# Autodesk Inventor assembly: Z18936-A FULL ASSEMBLY
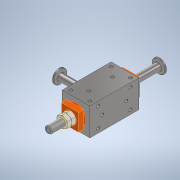
[picture p0: Inventor's stored thumbnail of the model, 180x180]
Saved by Autodesk Inventor 2021 (Build 250183000, 183)
## iProperties
Company: BROOKHAVEN NATIONAL LABORATORY
Created: 2019-11-05
Part Number: Z18936-A FULL ASSEMBLY
Description: ROTATING WATER JOINT SHAFT ASSEMBLY
Document SubType Name: Assembly
Designer: Work
Title: C:\Users\zconway\Documents\Inventor\HPR\Rotating Water Joint\Z18936-A FULL ASSEMBLY.stp
Author: zconway
Revision Number: 00
Sending System: Autodesk Inventor 2018
Preprocessor: ST-DEVELOPER v16.13
## Documents named in this file (9)
- C:\Users\Work\OneDrive - Brookhaven National Laboratory\Daniels, William intern HPR station\Arm\Z18936-A FULL ASSEMBLY.iam
- C:\Users\Work\OneDrive - Brookhaven National Laboratory\Daniels, William intern HPR station\Arm\Z18936-H HOUSING WELDMENT.iam
- C:\Users\Work\OneDrive - Brookhaven National Laboratory\Daniels, William intern HPR station\Arm\Z18936-S SHAFT ASSEMBLY.iam
- C:\Users\Work\OneDrive - Brookhaven National Laboratory\Daniels, William intern HPR station\Arm\Z18936-N1 COMPRESSION NUT.ipt
- C:\Users\Work\OneDrive - Brookhaven National Laboratory\Daniels, William intern HPR station\Arm\91907A140_TITANIUM THIN HEX NUT.ipt
- C:\Users\Work\OneDrive - Brookhaven National Laboratory\Daniels, William intern HPR station\Arm\8504A164_CORROSION-RESISTANT PRESS-FIT DRILL BUSHING.ipt
- C:\Users\Work\OneDrive - Brookhaven National Laboratory\Daniels, William intern HPR station\Arm\Z18936-B2 Shaft Gasket.ipt
- C:\Users\Work\OneDrive - Brookhaven National Laboratory\Daniels, William intern HPR station\Arm\Z18936-B1 THRUST PLATE.ipt
- C:\Users\Work\OneDrive - Brookhaven National Laboratory\Daniels, William intern HPR station\Arm\5908K150_ULTRA-CORROSION-RESISTANT SS BALL BEARING.ipt
## Components (13 placed, 8 different names)
1. Z18936-H HOUSING WELDMENT:1 [sub-assembly] — Rigid:5, Rigid:8, Rigid:12
2. Z18936-S SHAFT ASSEMBLY:1 [sub-assembly] — Rigid:7
3. Z18936-N1 COMPRESSION NUT:1 — Rigid:8
4. Z18936-N1 COMPRESSION NUT:2 — Rigid:5
5. 91907A140_TITANIUM THIN HEX NUT:1 — Rigid:3, Rigid:4
6. 91907A140_TITANIUM THIN HEX NUT:2 — Rigid:4
7. 8504A164_CORROSION-RESISTANT PRESS-FIT DRILL BUSHING:1 — Rigid:2, Rigid:3
8. Z18936-B2 Shaft Gasket:1 — Rigid:10, Rigid:11, Rigid:12
9. Z18936-B2 Shaft Gasket:2 — Rigid:9, Rigid:11
10. Z18936-B1 THRUST PLATE:1 — Rigid:6, Rigid:10
11. Z18936-B1 THRUST PLATE:2 — Rigid:1, Rigid:9
12. 5908K150_ULTRA-CORROSION-RESISTANT SS BALL BEARING:1 — Rigid:6, Rigid:7
13. 5908K150_ULTRA-CORROSION-RESISTANT SS BALL BEARING:2 — Rigid:1, Rigid:2
## Relationships (12: WeldJoint 12)
- Rigid:1 [WeldJoint]: Z18936-B1 THRUST PLATE:2 ↔ 5908K150_ULTRA-CORROSION-RESISTANT SS BALL BEARING:2
- Rigid:2 [WeldJoint]: 8504A164_CORROSION-RESISTANT PRESS-FIT DRILL BUSHING:1 ↔ 5908K150_ULTRA-CORROSION-RESISTANT SS BALL BEARING:2
- Rigid:3 [WeldJoint]: 91907A140_TITANIUM THIN HEX NUT:1 ↔ 8504A164_CORROSION-RESISTANT PRESS-FIT DRILL BUSHING:1
- Rigid:4 [WeldJoint]: 91907A140_TITANIUM THIN HEX NUT:1 ↔ 91907A140_TITANIUM THIN HEX NUT:2
- Rigid:5 [WeldJoint] (-3.81 mm): Z18936-H HOUSING WELDMENT:1 ↔ Z18936-N1 COMPRESSION NUT:2
- Rigid:6 [WeldJoint]: Z18936-B1 THRUST PLATE:1 ↔ 5908K150_ULTRA-CORROSION-RESISTANT SS BALL BEARING:1
- Rigid:7 [WeldJoint]: Z18936-S SHAFT ASSEMBLY:1 ↔ 5908K150_ULTRA-CORROSION-RESISTANT SS BALL BEARING:1
- Rigid:8 [WeldJoint] (-3.81 mm): Z18936-H HOUSING WELDMENT:1 ↔ Z18936-N1 COMPRESSION NUT:1
- Rigid:9 [WeldJoint]: Z18936-B2 Shaft Gasket:2 ↔ Z18936-B1 THRUST PLATE:2
- Rigid:10 [WeldJoint]: Z18936-B2 Shaft Gasket:1 ↔ Z18936-B1 THRUST PLATE:1
- Rigid:11 [WeldJoint] (19.431 mm): Z18936-B2 Shaft Gasket:1 ↔ Z18936-B2 Shaft Gasket:2
- Rigid:12 [WeldJoint]: Z18936-H HOUSING WELDMENT:1 ↔ Z18936-B2 Shaft Gasket:1
